# Autodesk Inventor assembly: PolarizationMethod
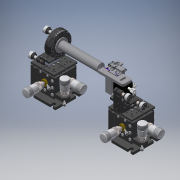
[picture p0: Inventor's stored thumbnail of the model, 180x180]
Saved by Autodesk Inventor 2019 (Build 230136000, 136)
## iProperties
Created: 2019-05-24
Part Number: PolarizationMethod
Document SubType Name: Assembly
Designer: aorfi
Author: aorfi
## Documents named in this file (11)
- C:\Users\aorfi\Documents\IQC\PolarizationMethod.iam
- C:\Users\aorfi\Documents\IQC\COTS\ThorLabs\3AxisStage-MBT616D.ipt
- C:\Users\aorfi\Documents\IQC\COTS\ThorLabs\RollStage-RSP1_M.ipt
- C:\Users\aorfi\Documents\IQC\COTS\ThorLabs\YawPitchStage-KM100PM.ipt
- C:\Users\aorfi\Documents\IQC\ChipMountAssembly.iam
- C:\Users\aorfi\Documents\IQC\CustomParts\FiberMount.ipt
- C:\Users\aorfi\Documents\IQC\CustomParts\FixedFiber.ipt
- C:\Users\aorfi\Documents\IQC\CustomParts\RubayetChip.ipt
- C:\Users\aorfi\Documents\IQC\COTS\ThorLabs\2StageDoveTail-DT12XY.ipt
- C:\Users\aorfi\Documents\IQC\CustomParts\AlignmentPiece.ipt
- C:\Users\aorfi\Documents\IQC\CustomParts\RemovableAlignmentPiece.ipt
## Components (13 placed, 10 different names)
1. 3AxisStage-MBT616D:1 — Mate:1, Flush:1, Mate:2, Flush:3, Flush:5
2. 3AxisStage-MBT616D:2 — Mate:6, Flush:4, Flush:5, Mate:8, Mate:12, Flush:7
3. RollStage-RSP1_M:1 — Mate:4, Angle:1, Mate:5, Mate:7, Mate:13, Mate:14
4. YawPitchStage-KM100PM:1 — Mate:2, Mate:4, Angle:1, Mate:13
5. ChipMountAssembly:1 [sub-assembly] — Mate:5, Mate:7
6. YawPitchStage-KM100PM:2 — Mate:8, Mate:12, Flush:7
7. FiberMount:1
8. FixedFiber:1
9. RubayetChip:1
10. RubayetChip:2
11. 2StageDoveTail-DT12XY:1
12. AlignmentPiece:1
13. RemovableAlignmentPiece:1
## Relationships (36: Mate 23, Flush 11, Angle 2)
- Mate:1: 3AxisStage-MBT616D:1
- Flush:1: 3AxisStage-MBT616D:1
- Mate:2: 3AxisStage-MBT616D:1 ↔ YawPitchStage-KM100PM:1
- Mate:4: RollStage-RSP1_M:1 ↔ YawPitchStage-KM100PM:1
- Flush:3: 3AxisStage-MBT616D:1
- Angle:1 (180 deg): RollStage-RSP1_M:1 ↔ YawPitchStage-KM100PM:1
- Mate:5: RollStage-RSP1_M:1 ↔ ChipMountAssembly:1
- Mate:6: 3AxisStage-MBT616D:2
- Flush:4: 3AxisStage-MBT616D:2
- Flush:5 (-200 mm): 3AxisStage-MBT616D:1 ↔ 3AxisStage-MBT616D:2
- Mate:7: RollStage-RSP1_M:1 ↔ ChipMountAssembly:1
- Mate:8: 3AxisStage-MBT616D:2 ↔ YawPitchStage-KM100PM:2
- Mate:12 (5 mm): 3AxisStage-MBT616D:2 ↔ YawPitchStage-KM100PM:2
- Flush:7: 3AxisStage-MBT616D:2 ↔ YawPitchStage-KM100PM:2
- Mate:13: RollStage-RSP1_M:1 ↔ YawPitchStage-KM100PM:1
- Mate:14: RollStage-RSP1_M:1
- [Flush] (-3 mm): YawPitchStage-KM100PM:2 ↔ 2StageDoveTail-DT12XY:1
- [Mate]: 2StageDoveTail-DT12XY:1
- [Mate]: YawPitchStage-KM100PM:2 ↔ FixedFiber:1
- [Mate]: FiberMount:1 ↔ RubayetChip:2
- [Mate]: FiberMount:1 ↔ RubayetChip:2
- [Flush]: FiberMount:1 ↔ RubayetChip:2
- [Mate]: FixedFiber:1 ↔ 2StageDoveTail-DT12XY:1
- [Mate]: FixedFiber:1 ↔ 2StageDoveTail-DT12XY:1
- [Angle] (180 deg): FixedFiber:1 ↔ 2StageDoveTail-DT12XY:1
- [Mate]: FixedFiber:1 ↔ RubayetChip:1
- [Mate]: FixedFiber:1 ↔ RubayetChip:1
- [Mate]: FixedFiber:1 ↔ AlignmentPiece:1
- [Flush]: FixedFiber:1 ↔ AlignmentPiece:1
- [Flush]: AlignmentPiece:1 ↔ RemovableAlignmentPiece:1
- [Flush]: FiberMount:1 ↔ RemovableAlignmentPiece:1
- [Flush]: AlignmentPiece:1 ↔ RemovableAlignmentPiece:1
- [Mate]: FiberMount:1 ↔ FixedFiber:1
- [Mate]: FiberMount:1 ↔ RemovableAlignmentPiece:1
- [Mate]: FiberMount:1 ↔ FixedFiber:1
- [Mate]: FixedFiber:1 ↔ RubayetChip:1
